# Autodesk Inventor assembly: Test_rig_assembly
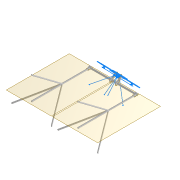
[picture p0: Inventor's stored thumbnail of the model, 180x180]
Saved by Autodesk Inventor 2022 (Build 260153000, 153)
## iProperties
Created: 2022-07-04
Part Number: Test_rig_assembly
Document SubType Name: Assembly
Designer: dell
Author: dell
## Documents named in this file (10)
- D:\xxxx\Uni\Part IV\MECHENG_700\Part_IV_project_CAD\Bird_skeleton_prototypes\Wing_drone_V1\Test_rig\Test_rig_assembly.iam
- D:\xxxx\Uni\Part IV\MECHENG_700\Part_IV_project_CAD\Bird_skeleton_prototypes\Wing_drone_V1\Test_rig\Aluminium_tube.ipt
- D:\xxxx\Uni\Part IV\MECHENG_700\Part_IV_project_CAD\Bird_skeleton_prototypes\Wing_drone_V1\Test_rig\Bearing.ipt
- D:\xxxx\Uni\Part IV\MECHENG_700\Part_IV_project_CAD\Bird_skeleton_prototypes\Wing_drone_V1\Test_rig\Test_tripod.ipt
- D:\xxxx\Uni\Part IV\MECHENG_700\Part_IV_project_CAD\Bird_skeleton_prototypes\Wing_drone_V1\Test_rig\Test_tripod_connector.ipt
- D:\xxxx\Uni\Part IV\MECHENG_700\Part_IV_project_CAD\Bird_skeleton_prototypes\Wing_drone_V1\Drone_assembly.iam
- D:\xxxx\Uni\Part IV\MECHENG_700\Part_IV_project_CAD\Bird_skeleton_prototypes\Wing_drone_V1\Test_rig\Bearing_housing.ipt
- D:\xxxx\Uni\Part IV\MECHENG_700\Part_IV_project_CAD\Bird_skeleton_prototypes\Wing_drone_V1\Test_rig\Bearing_fixing.ipt
- D:\xxxx\Uni\Part IV\MECHENG_700\Part_IV_project_CAD\Bird_skeleton_prototypes\Wing_drone_V1\Test_rig\Drone_mount.ipt
- D:\xxxx\Uni\Part IV\MECHENG_700\Part_IV_project_CAD\Bird_skeleton_prototypes\Wing_drone_V1\Test_rig\Aluminium_extrusion.ipt
## Components (20 placed, 9 different names)
1. Aluminium_tube:1 — Mate:7, Flush:3, Flush:4, Mate:8, Mate:9, Mate:14, Mate:28, Mate:30, Mate:32
2. Bearing:1 — Mate:8, Mate:10, Mate:11, Mate:12, Mate:13, Mate:15, Mate:29
3. Test_tripod:1 — Flush:1, Flush:2, Mate:1, Mate:2, Mate:3
4. Test_tripod:2 — Flush:1, Flush:2, Mate:4, Mate:5, Mate:6
5. Test_tripod_connector:2 — Mate:4, Mate:5, Mate:6, Flush:4
6. Test_tripod_connector:3 — Mate:1, Mate:2, Mate:3, Mate:7, Flush:3
7. Drone_assembly:1 [sub-assembly] — Mate:17, Mate:18, Mate:19, Mate:20, Mate:21, Mate:22
8. Bearing:2 — Mate:9, Mate:31, Mate:33, Mate:34, Mate:35, Mate:36, Mate:37
9. Bearing_housing:1 — Mate:10, Mate:13, Mate:16, Mate:24, Mate:25
10. Bearing_housing:2 — Mate:11, Mate:12, Mate:16, Mate:23
11. Bearing_fixing:1 — Mate:28, Mate:29
12. Bearing_fixing:2 — Mate:14, Mate:15
13. Drone_mount:1 — Mate:17, Mate:18, Mate:19, Mate:42, Mate:43
14. Drone_mount:2 — Mate:20, Mate:21, Mate:22, Mate:26, Mate:27, Flush:5
15. Aluminium_extrusion:1 — Mate:23, Mate:24, Mate:25, Mate:26, Mate:27, Flush:5
16. Bearing_fixing:3 — Mate:30, Mate:31
17. Bearing_fixing:4 — Mate:32, Mate:33
18. Bearing_housing:3 — Mate:34, Mate:37, Mate:39, Mate:40, Mate:41
19. Bearing_housing:4 — Mate:35, Mate:36
20. Aluminium_extrusion:2 — Mate:39, Mate:40, Mate:41, Mate:42, Mate:43
## Relationships (47: Mate 42, Flush 5)
- Flush:1: Test_tripod:1 ↔ Test_tripod:2
- Flush:2: Test_tripod:1 ↔ Test_tripod:2
- Mate:1: Test_tripod:1 ↔ Test_tripod_connector:3
- Mate:2 (-32 mm): Test_tripod:1 ↔ Test_tripod_connector:3
- Mate:3: Test_tripod:1 ↔ Test_tripod_connector:3
- Mate:4: Test_tripod:2 ↔ Test_tripod_connector:2
- Mate:5: Test_tripod:2 ↔ Test_tripod_connector:2
- Mate:6 (-32 mm): Test_tripod:2 ↔ Test_tripod_connector:2
- Mate:7: Aluminium_tube:1 ↔ Test_tripod_connector:3
- Flush:3: Aluminium_tube:1 ↔ Test_tripod_connector:3
- Flush:4: Aluminium_tube:1 ↔ Test_tripod_connector:2
- Mate:8: Aluminium_tube:1 ↔ Bearing:1
- Mate:9: Aluminium_tube:1 ↔ Bearing:2
- Mate:10: Bearing:1 ↔ Bearing_housing:1
- Mate:11: Bearing:1 ↔ Bearing_housing:2
- Mate:12: Bearing:1 ↔ Bearing_housing:2
- Mate:13: Bearing:1 ↔ Bearing_housing:1
- Mate:14: Aluminium_tube:1 ↔ Bearing_fixing:2
- Mate:15: Bearing:1 ↔ Bearing_fixing:2
- Mate:16: Bearing_housing:1 ↔ Bearing_housing:2
- Mate:17: Drone_assembly:1 ↔ Drone_mount:1
- Mate:18: Drone_assembly:1 ↔ Drone_mount:1
- Mate:19: Drone_assembly:1 ↔ Drone_mount:1
- Mate:20: Drone_assembly:1 ↔ Drone_mount:2
- Mate:21: Drone_assembly:1 ↔ Drone_mount:2
- Mate:22: Drone_assembly:1 ↔ Drone_mount:2
- Mate:23: Bearing_housing:2 ↔ Aluminium_extrusion:1
- Mate:24: Bearing_housing:1 ↔ Aluminium_extrusion:1
- Mate:25: Bearing_housing:1 ↔ Aluminium_extrusion:1
- Mate:26: Drone_mount:2 ↔ Aluminium_extrusion:1
- Mate:27: Drone_mount:2 ↔ Aluminium_extrusion:1
- Flush:5: Drone_mount:2 ↔ Aluminium_extrusion:1
- Mate:28: Aluminium_tube:1 ↔ Bearing_fixing:1
- Mate:29: Bearing:1 ↔ Bearing_fixing:1
- Mate:30: Aluminium_tube:1 ↔ Bearing_fixing:3
- Mate:31: Bearing:2 ↔ Bearing_fixing:3
- Mate:32: Aluminium_tube:1 ↔ Bearing_fixing:4
- Mate:33: Bearing:2 ↔ Bearing_fixing:4
- Mate:34: Bearing:2 ↔ Bearing_housing:3
- Mate:35: Bearing:2 ↔ Bearing_housing:4
- Mate:36: Bearing:2 ↔ Bearing_housing:4
- Mate:37: Bearing:2 ↔ Bearing_housing:3
- Mate:39: Bearing_housing:3 ↔ Aluminium_extrusion:2
- Mate:40: Bearing_housing:3 ↔ Aluminium_extrusion:2
- Mate:41: Bearing_housing:3 ↔ Aluminium_extrusion:2
- Mate:42: Drone_mount:1 ↔ Aluminium_extrusion:2
- Mate:43: Drone_mount:1 ↔ Aluminium_extrusion:2
